# Autodesk Inventor assembly: cellSTORM_v5_Alvium_dualcolour
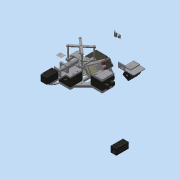
[picture p0: Inventor's stored thumbnail of the model, 180x180]
Saved by Autodesk Inventor 2019.4 (Build 234330000, 330)
## iProperties
Created: 2020-04-25
Part Number: cellSTORM_v5_Alvium_dualcolour
Document SubType Name: Assembly
Designer: diederichbenedict
Mass: 684.816 g
Surface Area: 2094.27 cm^2
Volume: 684.816 cm^3
Density: 1 g/cm^3
Author: diederichbenedict
## Documents named in this file (17)
- C:\Users\diederichbenedict\Dropbox\Dokumente\Promotion\PROJECTS\STORMoChip\GITHUB\CAD\cellSTORM_inverted\Workspace\cellSTORM_v5_inverted.iam
- C:\Users\diederichbenedict\Dropbox\Dokumente\Promotion\PROJECTS\STORMoChip\GITHUB\CAD\cellSTORM_inverted\Workspace\00_LASER_640nm.ipt
- C:\Users\diederichbenedict\Dropbox\Dokumente\Promotion\PROJECTS\STORMoChip\GITHUB\CAD\cellSTORM_inverted\Workspace\00_XY_stage-CHUO_SEIKI_LD-647-R1.iam
- C:\Users\diederichbenedict\Dropbox\Dokumente\Promotion\PROJECTS\STORMoChip\GITHUB\CAD\cellSTORM_inverted\Workspace\02_Nanoscopy_Chip.ipt
- C:\Users\diederichbenedict\Dropbox\Dokumente\Promotion\PROJECTS\STORMoChip\GITHUB\CAD\cellSTORM_inverted\Workspace\00_KES400.iam
- C:\Users\diederichbenedict\Dropbox\Dokumente\Promotion\PROJECTS\STORMoChip\GITHUB\CAD\cellSTORM_inverted\Workspace\00_Laser_532nm_200mw.ipt
- C:\Users\diederichbenedict\Dropbox\Dokumente\Promotion\PROJECTS\STORMoChip\GITHUB\CAD\cellSTORM_inverted\Workspace\cellSTORM_inverted_base_vß.ipt
- C:\Users\diederichbenedict\Dropbox\Dokumente\Promotion\PROJECTS\STORMoChip\GITHUB\CAD\cellSTORM_inverted\Workspace\cellSTORM_inverted_Laser_left.ipt
- C:\Users\diederichbenedict\Dropbox\Dokumente\Promotion\PROJECTS\STORMoChip\GITHUB\CAD\cellSTORM_inverted\Workspace\00_Rod_6mm_150mm.ipt
- C:\Users\diederichbenedict\Dropbox\Dokumente\Promotion\PROJECTS\STORMoChip\GITHUB\CAD\cellSTORM_inverted\Workspace\cellSTORM_inverted_sampleholder_bar.ipt
- C:\Users\diederichbenedict\Dropbox\Dokumente\Promotion\PROJECTS\STORMoChip\GITHUB\CAD\cellSTORM_inverted\Workspace\cellSTORM_inverted_sampleholder_bar_2.ipt
- C:\Users\diederichbenedict\Dropbox\Dokumente\Promotion\PROJECTS\STORMoChip\GITHUB\CAD\cellSTORM_inverted\Workspace\Assembly_cellSTORM_inverted_opticmodule_v0.iam
- C:\Users\diederichbenedict\Dropbox\Dokumente\Promotion\PROJECTS\STORMoChip\GITHUB\CAD\cellSTORM_inverted\Workspace\00_chip_01_old.ipt
- C:\Users\diederichbenedict\Dropbox\Dokumente\Promotion\PROJECTS\STORMoChip\GITHUB\CAD\cellSTORM_inverted\Workspace\cellSTORM_inverted_chiptray_oldchip_v0.ipt
- C:\Users\diederichbenedict\Dropbox\Dokumente\Promotion\PROJECTS\STORMoChip\GITHUB\CAD\cellSTORM_inverted\Workspace\cellSTORM_inverted_LED.ipt
- C:\Users\diederichbenedict\Dropbox\Dokumente\Promotion\PROJECTS\STORMoChip\GITHUB\CAD\cellSTORM_inverted\Workspace\Assembly_10x_Couplingscanner.iam
- C:\Users\diederichbenedict\Dropbox\Dokumente\Promotion\PROJECTS\STORMoChip\GITHUB\CAD\cellSTORM_inverted\Workspace\cellSTORM_inverted_chiptray_v0.ipt
## Components (22 placed, 16 different names)
1. 00_LASER_640nm:1
2. 02_Nanoscopy_Chip:1
3. 00_XY_stage-CHUO_SEIKI_LD-647-R1:2 [sub-assembly] — Mate:33, Flush:27, Mate:34
4. 00_XY_stage-CHUO_SEIKI_LD-647-R1:3 [sub-assembly] — Flush:28, Mate:35, Flush:29, Flush:35, Flush:36, Mate:69, Flush:48, Flush:49
5. 00_XY_stage-CHUO_SEIKI_LD-647-R1:4 [sub-assembly] — Flush:30, Mate:36, Mate:52, Mate:64, Flush:43, Flush:44
6. cellSTORM_inverted_base_vß:1 — Flush:35, Flush:36, Insert:25, Insert:26, Insert:27, Insert:28
7. 00_Rod_6mm_150mm:1 — Insert:25, Mate:65
8. 00_Rod_6mm_150mm:2 — Insert:28, Mate:55, Flush:45
9. 00_Rod_6mm_150mm:3 — Insert:26, Mate:66
10. 00_Rod_6mm_150mm:4 — Insert:27, Mate:54
11. cellSTORM_inverted_sampleholder_bar:1 — Mate:54, Mate:55, Flush:46
12. 00_chip_01_old:1 — Mate:67, Flush:47, Mate:68
13. cellSTORM_inverted_chiptray_v0:1
14. Assembly_cellSTORM_inverted_opticmodule_v0:1 [sub-assembly] — Mate:64, Flush:43, Flush:44
15. cellSTORM_inverted_LED:1 — Flush:45
16. cellSTORM_inverted_chiptray_oldchip_v0:2 — Insert:29, Insert:30, Mate:67, Flush:47, Mate:68
17. 00_Laser_532nm_200mw:1
18. cellSTORM_inverted_Laser_left:1
19. 00_LASER_640nm:2
20. 00_KES400:3 [sub-assembly]
21. cellSTORM_inverted_sampleholder_bar_2:1 — Mate:65, Mate:66, Flush:46, Insert:29, Insert:30
22. Assembly_10x_Couplingscanner:1 [sub-assembly] — Mate:69, Flush:48, Flush:49
## Relationships (32: Mate 13, Flush 13, Insert 6)
- Mate:33: 00_XY_stage-CHUO_SEIKI_LD-647-R1:2
- Flush:27: 00_XY_stage-CHUO_SEIKI_LD-647-R1:2
- Mate:34 (35 mm): 00_XY_stage-CHUO_SEIKI_LD-647-R1:2
- Flush:28: 00_XY_stage-CHUO_SEIKI_LD-647-R1:3
- Mate:35: 00_XY_stage-CHUO_SEIKI_LD-647-R1:3
- Flush:29 (35 mm): 00_XY_stage-CHUO_SEIKI_LD-647-R1:3
- Flush:30: 00_XY_stage-CHUO_SEIKI_LD-647-R1:4
- Mate:36: 00_XY_stage-CHUO_SEIKI_LD-647-R1:4
- Mate:52 (35 mm): 00_XY_stage-CHUO_SEIKI_LD-647-R1:4
- Flush:35: 00_XY_stage-CHUO_SEIKI_LD-647-R1:3 ↔ cellSTORM_inverted_base_vß:1
- Flush:36: 00_XY_stage-CHUO_SEIKI_LD-647-R1:3 ↔ cellSTORM_inverted_base_vß:1
- Insert:25: cellSTORM_inverted_base_vß:1 ↔ 00_Rod_6mm_150mm:1
- Insert:26: cellSTORM_inverted_base_vß:1 ↔ 00_Rod_6mm_150mm:3
- Insert:27: cellSTORM_inverted_base_vß:1 ↔ 00_Rod_6mm_150mm:4
- Insert:28: cellSTORM_inverted_base_vß:1 ↔ 00_Rod_6mm_150mm:2
- Mate:54: 00_Rod_6mm_150mm:4 ↔ cellSTORM_inverted_sampleholder_bar:1
- Mate:55: 00_Rod_6mm_150mm:2 ↔ cellSTORM_inverted_sampleholder_bar:1
- Mate:64: 00_XY_stage-CHUO_SEIKI_LD-647-R1:4 ↔ Assembly_cellSTORM_inverted_opticmodule_v0:1
- Flush:43: 00_XY_stage-CHUO_SEIKI_LD-647-R1:4 ↔ Assembly_cellSTORM_inverted_opticmodule_v0:1
- Flush:44: 00_XY_stage-CHUO_SEIKI_LD-647-R1:4 ↔ Assembly_cellSTORM_inverted_opticmodule_v0:1
- Flush:45: 00_Rod_6mm_150mm:2 ↔ cellSTORM_inverted_LED:1
- Mate:65: 00_Rod_6mm_150mm:1 ↔ cellSTORM_inverted_sampleholder_bar_2:1
- Mate:66: 00_Rod_6mm_150mm:3 ↔ cellSTORM_inverted_sampleholder_bar_2:1
- Flush:46: cellSTORM_inverted_sampleholder_bar:1 ↔ cellSTORM_inverted_sampleholder_bar_2:1
- Insert:29: cellSTORM_inverted_chiptray_oldchip_v0:2 ↔ cellSTORM_inverted_sampleholder_bar_2:1
- Insert:30: cellSTORM_inverted_chiptray_oldchip_v0:2 ↔ cellSTORM_inverted_sampleholder_bar_2:1
- Mate:67: 00_chip_01_old:1 ↔ cellSTORM_inverted_chiptray_oldchip_v0:2
- Flush:47 (-1 mm): 00_chip_01_old:1 ↔ cellSTORM_inverted_chiptray_oldchip_v0:2
- Mate:68 (1 mm): 00_chip_01_old:1 ↔ cellSTORM_inverted_chiptray_oldchip_v0:2
- Mate:69: 00_XY_stage-CHUO_SEIKI_LD-647-R1:3 ↔ Assembly_10x_Couplingscanner:1
- Flush:48: 00_XY_stage-CHUO_SEIKI_LD-647-R1:3 ↔ Assembly_10x_Couplingscanner:1
- Flush:49: 00_XY_stage-CHUO_SEIKI_LD-647-R1:3 ↔ Assembly_10x_Couplingscanner:1
## Named parameters: d_1 = 35 mm
